# Autodesk Inventor assembly: リンク_6_1
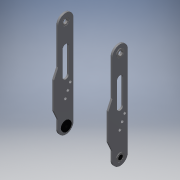
[picture p0: Inventor's stored thumbnail of the model, 180x180]
Saved by Autodesk Inventor 2018 (Build 220112000, 112)
## iProperties
Created: 2016-08-23
Part Number: リンク_6_1
Material: 一般
Document SubType Name: Assembly
Designer: hiro
Mass: 25.4181 g
Surface Area: 148.711 cm^2
Volume: 11.4997 cm^3
Density: 2.21034 g/cm^3
Author: hiro
## Documents named in this file (4)
- C:\Users\taka\Documents\github\OpenPlatform\mechanism\OpenPlatform_ver1_0\下半身_160823\リンク\リンク_6_1.iam
- C:\Users\taka\Documents\github\OpenPlatform\mechanism\OpenPlatform_ver1_0\既製品\NSK_RB_MF85ZZ\MF85ZZ.iam
- C:\Users\taka\Documents\github\OpenPlatform\mechanism\OpenPlatform_ver1_0\下半身\リンク\スペーサ\足首_スペーサ_1_1.ipt
- C:\Users\taka\Documents\github\OpenPlatform\mechanism\OpenPlatform_ver1_0\下半身_160823\リンク\リンク_メインフレーム_6_3.ipt
## Components (8 placed, 3 different names)
1. MF85ZZ:1 [sub-assembly] — 挿入:28
2. MF85ZZ:2 [sub-assembly] — 挿入:27
3. 足首_スペーサ_1_1:1
4. 足首_スペーサ_1_1:2
5. MF85ZZ:3 [sub-assembly] — 挿入:29
6. MF85ZZ:4 [sub-assembly] — 挿入:26
7. リンク_メインフレーム_6_3:1 — 挿入:28, 挿入:29
8. リンク_メインフレーム_6_3:2 — 挿入:26, 挿入:27
## Relationships (4: Insert 4)
- 挿入:26 [Insert]: MF85ZZ:4 ↔ リンク_メインフレーム_6_3:2
- 挿入:27 [Insert]: MF85ZZ:2 ↔ リンク_メインフレーム_6_3:2
- 挿入:28 [Insert]: MF85ZZ:1 ↔ リンク_メインフレーム_6_3:1
- 挿入:29 [Insert]: MF85ZZ:3 ↔ リンク_メインフレーム_6_3:1
